# Autodesk Inventor assembly: Мехатрон Сборка1
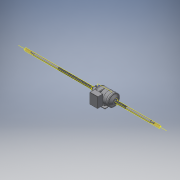
[picture p0: Inventor's stored thumbnail of the model, 180x180]
Saved by Autodesk Inventor 2016 SP1 (Build 200210100, 210)
## iProperties
Created: 2016-04-25
Part Number: Мехатрон Сборка1
Material: Типовые
Document SubType Name: Assembly
Designer: AS
Author: AS
## Documents named in this file (11)
- H:\Projects\GitHub\mechatron\Мехатрон Сборка1.iam
- H:\Projects\GitHub\mechatron\Vint.ipt
- H:\Projects\GitHub\mechatron\1 Корпус.ipt
- H:\Projects\GitHub\mechatron\2 крышка.ipt
- H:\Projects\GitHub\mechatron\Деталь 3.ipt
- H:\Projects\GitHub\mechatron\Деталь 4.ipt
- H:\Projects\GitHub\mechatron\Деталь 5.ipt
- H:\Projects\GitHub\mechatron\Деталь 6.ipt
- H:\Projects\GitHub\mechatron\Полый вал.ipt
- H:\Projects\GitHub\mechatron\Крышка контейнера.ipt
- H:\Projects\GitHub\mechatron\Мехатрон Сборка1\Мастер проектирования\Болтовое соединение3.iam
## Components (13 placed, 10 different names)
1. Vint:1 — Совмещение:1
2. 1 Корпус:1 — Совмещение:2, Заподлицо:3, Заподлицо:9, Заподлицо:10, Заподлицо:11, Совмещение:8, Совмещение:13, Совмещение:14
3. 2 крышка:1 — Заподлицо:2, Совмещение:3, Совмещение:12, Совмещение:13
4. Деталь 3:1 — Заподлицо:4, Совмещение:4, Совмещение:14, Совмещение:15
5. Деталь 4:1 — Заподлицо:5, Совмещение:5, Совмещение:7, Совмещение:15, Совмещение:16
6. Деталь 5:1 — Заподлицо:6, Совмещение:6, Совмещение:9, Вставка:1, Совмещение:10, Совмещение:11, Совмещение:12
7. Деталь 6:1 — Заподлицо:7, Совмещение:7, Совмещение:16
8. Полый вал:1 — Заподлицо:8, Совмещение:9, Вставка:1
9. Крышка контейнера:1 — Заподлицо:10, Заподлицо:11, Совмещение:8
10. Болтовое соединение:1 [sub-assembly] — Совмещение:10, Совмещение:11
11. Болтовое соединение:2 [sub-assembly]
12. Болтовое соединение:3 [sub-assembly]
13. Болтовое соединение:4 [sub-assembly]
## Component patterns: (4 elements, first: Болтовое соединение:1)
## Relationships (27: Mate 16, Flush 10, Insert 1)
- Совмещение:1 [Mate]: Vint:1
- Заподлицо:2 [Flush]: 2 крышка:1
- Совмещение:2 [Mate]: 1 Корпус:1
- Совмещение:3 [Mate]: 2 крышка:1
- Заподлицо:3 [Flush]: 1 Корпус:1
- Заподлицо:4 [Flush]: Деталь 3:1
- Совмещение:4 [Mate]: Деталь 3:1
- Заподлицо:5 [Flush]: Деталь 4:1
- Совмещение:5 [Mate]: Деталь 4:1
- Заподлицо:6 [Flush]: Деталь 5:1
- Совмещение:6 [Mate]: Деталь 5:1
- Заподлицо:7 [Flush]: Деталь 6:1
- Совмещение:7 [Mate]: Деталь 4:1 ↔ Деталь 6:1
- Заподлицо:8 [Flush]: Полый вал:1
- Заподлицо:9 [Flush]: 1 Корпус:1
- Заподлицо:10 [Flush]: 1 Корпус:1 ↔ Крышка контейнера:1
- Заподлицо:11 [Flush]: 1 Корпус:1 ↔ Крышка контейнера:1
- Совмещение:8 [Mate]: 1 Корпус:1 ↔ Крышка контейнера:1
- Совмещение:9 [Mate]: Деталь 5:1 ↔ Полый вал:1
- Вставка:1 [Insert]: Деталь 5:1 ↔ Полый вал:1
- Совмещение:10 [Mate]: Деталь 5:1 ↔ Болтовое соединение:1
- Совмещение:11 [Mate]: Деталь 5:1 ↔ Болтовое соединение:1
- Совмещение:12 [Mate]: 2 крышка:1 ↔ Деталь 5:1
- Совмещение:13 [Mate]: 1 Корпус:1 ↔ 2 крышка:1
- Совмещение:14 [Mate]: 1 Корпус:1 ↔ Деталь 3:1
- Совмещение:15 [Mate]: Деталь 3:1 ↔ Деталь 4:1
- Совмещение:16 [Mate]: Деталь 4:1 ↔ Деталь 6:1
